# Autodesk Inventor assembly: Ensamblaje1
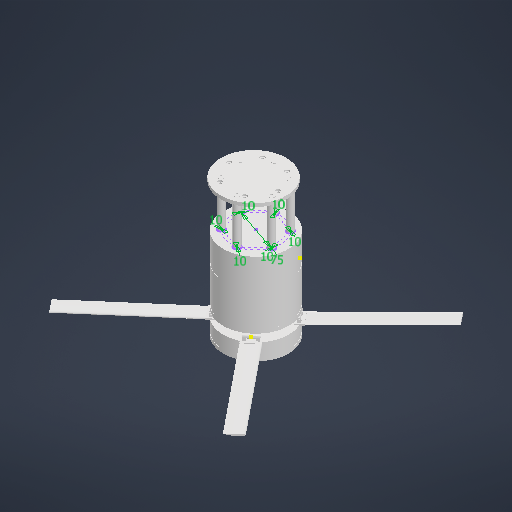
[picture p0: Inventor's stored thumbnail of the model, 512x512]
Saved by Autodesk Inventor 2026.1 (Build 301233000, 233)
## iProperties
Created: 2025-09-15
Part Number: Ensamblaje1
Document SubType Name: Assembly
Designer: Usuario
Author: Usuario
## Documents named in this file (11)
- C:\Users\Usuario\Desktop\Cansat\Cansat 2\Ensamblaje1.iam
- C:\Users\Usuario\Desktop\Cansat\Cansat 2\Pieza1.ipt
- C:\Users\Usuario\Desktop\Cansat\Cansat 2\Pieza2.ipt
- C:\Users\Usuario\Desktop\Cansat\Cansat 2\Pieza4.ipt
- C:\Users\Usuario\Desktop\Cansat\Cansat 2\Pieza3.ipt
- C:\Users\Usuario\Desktop\Cansat\Cansat 2\Pieza6.ipt
- C:\Users\Usuario\Documents\Inventor\Content Center Files\R2026\es-ES\GB_T 276-94 60000-2RS and 2LS\Bearing 6000-2RS GB_T 276-94.ipt
- C:\Users\Usuario\Desktop\Cansat\Cansat 2\Pieza5.ipt
- C:\Users\Usuario\Desktop\Cansat\Cansat 2\Pieza7.ipt
- C:\Users\Usuario\Desktop\Cansat\Cansat 2\Pieza8.ipt
- C:\Users\Usuario\Desktop\Cansat\Cansat 2\Pieza9.ipt
## Components (13 placed, 10 different names)
1. Pieza1:1 — Insertar:1
2. Pieza2:1 — Insertar:1, Insertar:2
3. Pieza4:1 — Insertar:3, Insertar:5
4. Pieza3:1 — Insertar:2, Insertar:4
5. Pieza6:1 — Coincidencia:1, De rotación:1, Insertar:7, Insertar:8, Insertar:9, Insertar:10
6. Rolling bearing GB/T 276-1994 Type 60000-2RS and 2LS 6000-2RS:1 — Coincidencia:1, De rotación:1, Insertar:3, Insertar:4
7. Pieza5:1 — Insertar:5, Insertar:6
8. Pieza7:1 — Insertar:6
9. Pieza8:1
10. Pieza9:1 — Insertar:10
11. Pieza9:2 — Insertar:9
12. Pieza9:3 — Insertar:8
13. Pieza9:4 — Insertar:7
## Relationships (12: Insert 10, Mate 1, RevoluteJoint 1)
- Insertar:1: Pieza1:1 ↔ Pieza2:1
- Insertar:2: Pieza2:1 ↔ Pieza3:1
- Coincidencia:1 [Mate]: Pieza6:1 ↔ Rolling bearing GB/T 276-1994 Type 60000-2RS and 2LS 6000-2RS:1
- De rotación:1 [RevoluteJoint]: Pieza6:1 ↔ Rolling bearing GB/T 276-1994 Type 60000-2RS and 2LS 6000-2RS:1
- Insertar:3: Pieza4:1 ↔ Rolling bearing GB/T 276-1994 Type 60000-2RS and 2LS 6000-2RS:1
- Insertar:4: Pieza3:1 ↔ Rolling bearing GB/T 276-1994 Type 60000-2RS and 2LS 6000-2RS:1
- Insertar:5: Pieza4:1 ↔ Pieza5:1
- Insertar:6: Pieza5:1 ↔ Pieza7:1
- Insertar:7: Pieza6:1 ↔ Pieza9:4
- Insertar:8: Pieza6:1 ↔ Pieza9:3
- Insertar:9: Pieza6:1 ↔ Pieza9:2
- Insertar:10: Pieza6:1 ↔ Pieza9:1
